# Autodesk Inventor assembly: Mecanismo Modelado
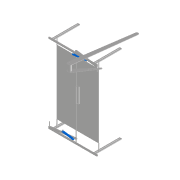
[picture p0: Inventor's stored thumbnail of the model, 180x180]
Saved by Autodesk Inventor 2021 (Build 250183000, 183)
## iProperties
Created: 2021-04-19
Part Number: Mecanismo Modelado
Document SubType Name: Assembly
Designer: carlo
Author: carlo
## Documents named in this file (10)
- C:\Users\carlo\Desktop\Concepto\Modelado Mecanismo\Mecanismo Modelado.iam
- C:\Users\carlo\Desktop\Concepto\Modelado Mecanismo\Bancada.ipt
- C:\Users\carlo\Desktop\Concepto\Modelado Mecanismo\Eslabon1.ipt
- C:\Users\carlo\Desktop\Concepto\Modelado Mecanismo\Eslabon2.ipt
- C:\Users\carlo\Desktop\Concepto\Modelado Mecanismo\Palanca.ipt
- C:\Users\carlo\Desktop\Concepto\Modelado Mecanismo\pin5.ipt
- C:\Users\carlo\Desktop\Concepto\Modelado Mecanismo\pin10.ipt
- C:\Users\carlo\Desktop\Concepto\Modelado Mecanismo\pin5corto.ipt
- C:\Users\carlo\Desktop\Concepto\Modelado Mecanismo\union.ipt
- C:\Users\carlo\Desktop\Concepto\Modelado Mecanismo\Bandeja.ipt
## Components (16 placed, 9 different names)
1. Bancada:1 — Coincidencia:1, Tangente:1, Nivelación:2, Cilíndrica:5, Nivelación:7, Nivelación:12, Coincidencia:7, Tangente:3, Tangente:4, Nivelación:14
2. Eslabon1:1 — Coincidencia:1, Coincidencia:2, Cilíndrica:6, Cilíndrica:7
3. Eslabon2:1 — Cilíndrica:4, Coincidencia:2, Coincidencia:3, Cilíndrica:8, Nivelación:6, Cilíndrica:14, Nivelación:13
4. Palanca:1 — Coincidencia:3, Coincidencia:4, Nivelación:5
5. pin10:1 — Coincidencia:4, Nivelación:5
6. pin5:4 — Cilíndrica:4, Tangente:1, Nivelación:2
7. pin5corto:1 — Cilíndrica:5, Cilíndrica:6, Nivelación:7
8. pin5corto:2 — Cilíndrica:7, Cilíndrica:8, Nivelación:6
9. Bancada:2 — Coincidencia:5, Nivelación:9, Tangente:2, Nivelación:10, Cilíndrica:11, Nivelación:12, Coincidencia:7
10. Eslabon1:2 — Coincidencia:5, Coincidencia:6, Cilíndrica:10, Cilíndrica:13
11. Eslabon2:2 — Coincidencia:6, Nivelación:11, Cilíndrica:9, Cilíndrica:12, Cilíndrica:15
12. pin5:5 — Nivelación:9, Tangente:2, Cilíndrica:9
13. pin5corto:3 — Nivelación:10, Cilíndrica:10, Cilíndrica:11
14. pin5corto:4 — Nivelación:11, Cilíndrica:12, Cilíndrica:13
15. union:1 — Cilíndrica:14, Cilíndrica:15, Cilíndrica:16, Nivelación:13
16. Bandeja:1 — Cilíndrica:16, Tangente:3, Tangente:4, Nivelación:14
## Relationships (34: CylindricalJoint 13, Flush 10, Mate 7, Tangent 4)
- Coincidencia:1 [Mate] (10 mm): Bancada:1 ↔ Eslabon1:1
- Cilíndrica:4 [CylindricalJoint]: Eslabon2:1 ↔ pin5:4
- Tangente:1: Bancada:1 ↔ pin5:4
- Coincidencia:2 [Mate] (3 mm): Eslabon1:1 ↔ Eslabon2:1
- Nivelación:2 [Flush]: Bancada:1 ↔ pin5:4
- Coincidencia:3 [Mate] (10 mm): Eslabon2:1 ↔ Palanca:1
- Coincidencia:4 [Mate]: Palanca:1 ↔ pin10:1
- Nivelación:5 [Flush]: Palanca:1 ↔ pin10:1
- Cilíndrica:5 [CylindricalJoint]: Bancada:1 ↔ pin5corto:1
- Cilíndrica:6 [CylindricalJoint]: Eslabon1:1 ↔ pin5corto:1
- Cilíndrica:7 [CylindricalJoint]: Eslabon1:1 ↔ pin5corto:2
- Cilíndrica:8 [CylindricalJoint]: Eslabon2:1 ↔ pin5corto:2
- Nivelación:6 [Flush] (-1 mm): Eslabon2:1 ↔ pin5corto:2
- Nivelación:7 [Flush]: Bancada:1 ↔ pin5corto:1
- Coincidencia:5 [Mate] (10 mm): Bancada:2 ↔ Eslabon1:2
- Coincidencia:6 [Mate] (3 mm): Eslabon1:2 ↔ Eslabon2:2
- Nivelación:9 [Flush]: Bancada:2 ↔ pin5:5
- Tangente:2: Bancada:2 ↔ pin5:5
- Nivelación:10 [Flush]: Bancada:2 ↔ pin5corto:3
- Nivelación:11 [Flush] (-1 mm): Eslabon2:2 ↔ pin5corto:4
- Cilíndrica:9 [CylindricalJoint]: Eslabon2:2 ↔ pin5:5
- Cilíndrica:10 [CylindricalJoint]: Eslabon1:2 ↔ pin5corto:3
- Cilíndrica:11 [CylindricalJoint]: Bancada:2 ↔ pin5corto:3
- Cilíndrica:12 [CylindricalJoint]: Eslabon2:2 ↔ pin5corto:4
- Cilíndrica:13 [CylindricalJoint]: Eslabon1:2 ↔ pin5corto:4
- Nivelación:12 [Flush]: Bancada:1 ↔ Bancada:2
- Coincidencia:7 [Mate] (517.58 mm): Bancada:1 ↔ Bancada:2
- Cilíndrica:14 [CylindricalJoint]: Eslabon2:1 ↔ union:1
- Cilíndrica:15 [CylindricalJoint]: Eslabon2:2 ↔ union:1
- Cilíndrica:16 [CylindricalJoint]: union:1 ↔ Bandeja:1
- Nivelación:13 [Flush]: Eslabon2:1 ↔ union:1
- Tangente:3: Bancada:1 ↔ Bandeja:1
- Tangente:4: Bancada:1 ↔ Bandeja:1
- Nivelación:14 [Flush] (50 mm): Bancada:1 ↔ Bandeja:1
